# Autodesk Inventor assembly: robot
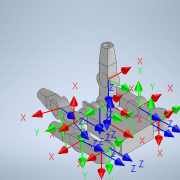
[picture p0: Inventor's stored thumbnail of the model, 180x180]
Saved by Autodesk Inventor 2020.2 (Build 242310000, 310)
## iProperties
Created: 2021-01-29
Part Number: robot
Document SubType Name: Assembly
Designer: DELL
Author: DELL
## Documents named in this file (5)
- D:\repo\FlexipodHardware\Flexipod2.0\Cadquery_module\v8.0\robot.iam
- D:\repo\FlexipodHardware\Flexipod2.0\Cadquery_module\v8.0\body.ipt
- D:\repo\FlexipodHardware\Flexipod2.0\Cadquery_module\v8.0\hip.ipt
- D:\repo\FlexipodHardware\Flexipod2.0\Cadquery_module\v8.0\thigh.ipt
- D:\repo\FlexipodHardware\Flexipod2.0\Cadquery_module\v8.0\shank.ipt
## Components (13 placed, 4 different names)
1. body:1 — Flush:1, Flush:2, Flush:3, Mate:1, Mate:2, Mate:3, Mate:4, Mate:5, Mate:6, Mate:7, Mate:8, Angle:1, Angle:2, Angle:3, Angle:4
2. hip:1 — Mate:3, Mate:4, Angle:2, Mate:10, Mate:14
3. hip:2 — Mate:1, Mate:2, Angle:1, Mate:9, Flush:4
4. hip:3 — Mate:7, Mate:8, Angle:4, Mate:12, Flush:5
5. hip:4 — Mate:5, Mate:6, Angle:3, Mate:11, Mate:13
6. thigh:1 — Mate:9, Flush:4, Mate:15, Mate:20
7. thigh:2 — Mate:10, Mate:14, Mate:17, Flush:7
8. thigh:3 — Mate:11, Mate:13, Mate:16, Flush:6
9. thigh:4 — Mate:12, Flush:5, Mate:18, Mate:19
10. shank:1 — Mate:16, Flush:6
11. shank:2 — Mate:15, Mate:20
12. shank:3 — Mate:17, Flush:7
13. shank:4 — Mate:18, Mate:19
## Relationships (31: Mate 20, Flush 7, Angle 4)
- Flush:1: body:1
- Flush:2: body:1
- Flush:3: body:1
- Mate:1: body:1 ↔ hip:2
- Mate:2: body:1 ↔ hip:2
- Mate:3: body:1 ↔ hip:1
- Mate:4: body:1 ↔ hip:1
- Mate:5: body:1 ↔ hip:4
- Mate:6: body:1 ↔ hip:4
- Mate:7: body:1 ↔ hip:3
- Mate:8: body:1 ↔ hip:3
- Angle:1 (90 deg): body:1 ↔ hip:2
- Angle:2 (90 deg): body:1 ↔ hip:1
- Angle:3 (90 deg): body:1 ↔ hip:4
- Angle:4 (-180 deg): body:1 ↔ hip:3
- Mate:9: hip:2 ↔ thigh:1
- Mate:10: hip:1 ↔ thigh:2
- Mate:11: hip:4 ↔ thigh:3
- Mate:12: hip:3 ↔ thigh:4
- Flush:4: hip:2 ↔ thigh:1
- Mate:13: hip:4 ↔ thigh:3
- Flush:5: hip:3 ↔ thigh:4
- Mate:14: hip:1 ↔ thigh:2
- Mate:15: thigh:1 ↔ shank:2
- Mate:16: thigh:3 ↔ shank:1
- Mate:17: thigh:2 ↔ shank:3
- Mate:18: thigh:4 ↔ shank:4
- Mate:19: thigh:4 ↔ shank:4
- Flush:6: thigh:3 ↔ shank:1
- Flush:7: thigh:2 ↔ shank:3
- Mate:20: thigh:1 ↔ shank:2
